# Autodesk Inventor assembly: track
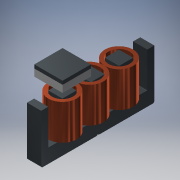
[picture p0: Inventor's stored thumbnail of the model, 180x180]
Saved by Autodesk Inventor 2019 (Build 230136000, 136)
## iProperties
Created: 2021-07-12
Part Number: track
Document SubType Name: Assembly
Designer: pensun
Author: pensun
## Documents named in this file (5)
- C:\Pengpeng\02 coreWithCoil(Ecore)\Hyperloop\Track\track.iam
- C:\Pengpeng\02 coreWithCoil(Ecore)\Hyperloop\E core\Ecore.ipt
- C:\Pengpeng\02 coreWithCoil(Ecore)\Hyperloop\Coil\coil.ipt
- C:\Pengpeng\02 coreWithCoil(Ecore)\Hyperloop\plate\al.ipt
- C:\Pengpeng\02 coreWithCoil(Ecore)\Hyperloop\plate\Iron.ipt
## Components (5 placed, 4 different names)
1. coil:1 — Mate:1
2. al:1 — Mate:2, Flush:1, Flush:2, Mate:3
3. Iron:1 — Mate:2, Flush:1, Flush:2
4. Ecore:1
5. Ecore:2 — Mate:1, Mate:3
## Component patterns: (2 elements, first: Ecore:1)
## Relationships (5: Mate 3, Flush 2)
- Mate:1: coil:1 ↔ Ecore:2
- Mate:2: al:1 ↔ Iron:1
- Flush:1: al:1 ↔ Iron:1
- Flush:2: al:1 ↔ Iron:1
- Mate:3 (15 mm): al:1 ↔ Ecore:2
